# Autodesk Inventor assembly: EngineComplete
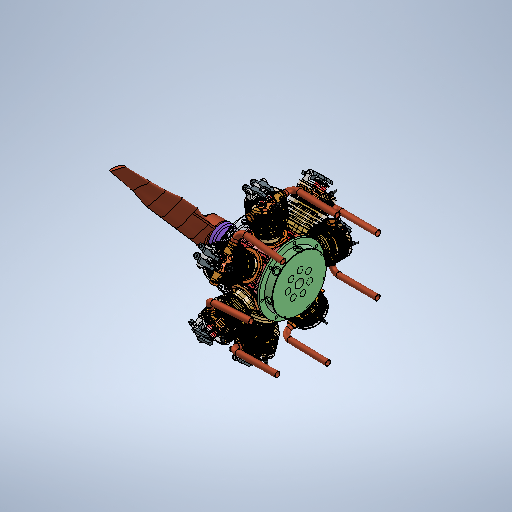
[picture p0: Inventor's stored thumbnail of the model, 512x512]
Saved by Autodesk Inventor 2025 (Build 290162010, 162A)
## iProperties
Created: 2024-07-16
Part Number: EngineComplete
Document SubType Name: Assembly
Designer: ffogue
Author: ffogue
## Documents named in this file (15)
- C:\Users\Fabri\Documents\Inventor\Stermotor\EngineComplete.iam
- C:\Users\Fabri\Documents\Inventor\Stermotor\Zylinder.ipt
- C:\Users\Fabri\Documents\Inventor\Stermotor\MotorBlock_First.iam
- C:\Users\Fabri\Documents\Inventor\Stermotor\pleuel.ipt
- C:\Users\Fabri\Documents\Inventor\Stermotor\Kolben.iam
- C:\Users\Fabri\Documents\Inventor\Stermotor\MotorBlock.iam
- C:\Users\Fabri\Documents\Inventor\Stermotor\sonnenrad.ipt
- C:\Users\Fabri\Documents\Inventor\Stermotor\Decke_grün.ipt
- C:\Users\Fabri\Documents\Inventor\Stermotor\Cylinder.iam
- C:\Users\Fabri\Documents\Inventor\Stermotor\VenturiEinsatz.ipt
- C:\Users\Fabri\Documents\Inventor\Stermotor\zylinderfussdichtung.ipt
- C:\Users\Fabri\Documents\Inventor\Stermotor\Aschse.iam
- C:\Users\Fabri\Documents\Inventor\Stermotor\PlanetenRad.ipt
- C:\Users\Fabri\Documents\Inventor\Stermotor\Stirnzahnrad12.ipt
- C:\Users\Fabri\Documents\Inventor\Stermotor\Rad16_5.ipt
## Components (47 placed, 13 different names)
1. Zylinder:1 — Mate:1, Mate:2, Insert:1, Mate:4, Mate:8, Mate:10, Mate:11, Mate:12, Mate:13, Insert:10, Mate:30, Insert:14, Mate:39, Insert:18, Insert:19, Insert:20, Insert:21, Insert:22, Insert:23, Mate:50, Insert:28
2. MotorBlock_First:1 [sub-assembly] — Mate:2, Insert:1, Mate:5, Insert:2, Mate:7, Insert:3, Mate:14, Insert:4, Mate:16, Insert:5, Mate:18, Insert:6, Mate:20, Insert:7, Mate:28, Insert:12, Insert:29
3. Kolben:1 [sub-assembly] — Mate:4, Mate:6, Mate:26
4. pleuel:1 — Mate:5, Insert:2, Mate:6
5. pleuel:3 — Mate:7, Insert:3, Mate:9
6. Kolben:3 [sub-assembly] — Mate:8, Mate:9, Mate:44
7. Kolben:4 [sub-assembly] — Mate:10, Mate:15, Mate:43
8. Kolben:5 [sub-assembly] — Mate:11, Mate:17, Mate:42
9. Kolben:6 [sub-assembly] — Mate:12, Mate:19, Mate:41
10. Kolben:7 [sub-assembly] — Mate:13, Mate:21, Mate:40
11. pleuel:4 — Mate:14, Mate:15, Insert:4
12. pleuel:5 — Mate:16, Mate:17, Insert:5
13. pleuel:6 — Mate:18, Insert:6, Mate:19
14. pleuel:7 — Mate:20, Insert:7, Mate:21
15. sonnenrad:1 — Mate:30, Insert:14, Mate:38
16. Decke_grün:1 — Mate:34, Mate:38, Mate:39, Insert:17, Insert:18, Mate:53
17. MotorBlock:2 [sub-assembly] — Mate:28, Insert:12
18. MotorBlock:1 [sub-assembly] — Mate:27, Insert:11
19. Cylinder:1 [sub-assembly] — Mate:26, Mate:27, Insert:10, Insert:11
20. Cylinder:2 [sub-assembly] — Mate:40, Insert:19, Mate:45, Insert:24
21. Cylinder:3 [sub-assembly] — Mate:41, Insert:20, Mate:46, Insert:25
22. Cylinder:4 [sub-assembly] — Mate:42, Insert:21, Mate:47, Insert:26
23. Cylinder:5 [sub-assembly] — Mate:43, Insert:22, Mate:48, Insert:27
24. Cylinder:6 [sub-assembly] — Mate:44, Insert:23, Mate:49
25. MotorBlock:3 [sub-assembly] — Mate:49
26. MotorBlock:4 [sub-assembly] — Mate:48, Insert:27
27. MotorBlock:5 [sub-assembly] — Mate:47, Insert:26
28. MotorBlock:6 [sub-assembly] — Mate:46, Insert:25
29. MotorBlock:7 [sub-assembly] — Mate:45, Insert:24
30. Aschse:1 [sub-assembly] — Rotation:2, Mate:53, Insert:29, Mate:54, Insert:30
31. Stirnzahnrad1:1 — Mate:52, Flush:1, Rotation:1, Flush:2, Rotation:4
32. Stirnzahnrad1:2 — Mate:52, Flush:1, Rotation:1, Rotation:2, Main Motion, Rotation:3, Tangent:2, Mate:54, Insert:30
33. Stirnzahnrad2:1 — Flush:2, Rotation:3, Tangent:2, Rotation:4
34. VenturiEinsatz:2 — Mate:34, Insert:17
35. VenturiEinsatz:3
36. VenturiEinsatz:4
37. VenturiEinsatz:5
38. VenturiEinsatz:6
39. VenturiEinsatz:7
40. VenturiEinsatz:8
41. zylinderfussdichtung:1 — Mate:50, Insert:28
42. zylinderfussdichtung:2
43. zylinderfussdichtung:3
44. zylinderfussdichtung:4
45. zylinderfussdichtung:5
46. zylinderfussdichtung:6
47. zylinderfussdichtung:7
## Component patterns: (7 elements, first: VenturiEinsatz:2), (7 elements, first: zylinderfussdichtung:1)
## Relationships (74: Mate 41, Insert 25, RelateRotation 4, Flush 2, Angle 1, Tangent 1)
- Mate:1: Zylinder:1
- Mate:2: Zylinder:1 ↔ MotorBlock_First:1
- Insert:1: Zylinder:1 ↔ MotorBlock_First:1
- Mate:4: Zylinder:1 ↔ Kolben:1
- Mate:5: MotorBlock_First:1 ↔ pleuel:1
- Insert:2: MotorBlock_First:1 ↔ pleuel:1
- Mate:6: Kolben:1 ↔ pleuel:1
- Mate:7: MotorBlock_First:1 ↔ pleuel:3
- Insert:3: MotorBlock_First:1 ↔ pleuel:3
- Mate:8: Zylinder:1 ↔ Kolben:3
- Mate:9: pleuel:3 ↔ Kolben:3
- Mate:10: Zylinder:1 ↔ Kolben:4
- Mate:11: Zylinder:1 ↔ Kolben:5
- Mate:12: Zylinder:1 ↔ Kolben:6
- Mate:13: Zylinder:1 ↔ Kolben:7
- Mate:14: MotorBlock_First:1 ↔ pleuel:4
- Mate:15: Kolben:4 ↔ pleuel:4
- Insert:4: MotorBlock_First:1 ↔ pleuel:4
- Mate:16: MotorBlock_First:1 ↔ pleuel:5
- Mate:17: Kolben:5 ↔ pleuel:5
- Insert:5: MotorBlock_First:1 ↔ pleuel:5
- Mate:18: MotorBlock_First:1 ↔ pleuel:6
- Insert:6: MotorBlock_First:1 ↔ pleuel:6
- Mate:19: Kolben:6 ↔ pleuel:6
- Mate:20: MotorBlock_First:1 ↔ pleuel:7
- Insert:7: MotorBlock_First:1 ↔ pleuel:7
- Mate:21: Kolben:7 ↔ pleuel:7
- Mate:26: Kolben:1 ↔ Cylinder:1
- Mate:27: MotorBlock:1 ↔ Cylinder:1
- Insert:10 (-5.5 mm): Zylinder:1 ↔ Cylinder:1
- Insert:11: MotorBlock:1 ↔ Cylinder:1
- Mate:28: MotorBlock_First:1 ↔ MotorBlock:2
- Insert:12: MotorBlock_First:1 ↔ MotorBlock:2
- Mate:30: Zylinder:1 ↔ sonnenrad:1
- Insert:14: Zylinder:1 ↔ sonnenrad:1
- Mate:34: Decke_grün:1 ↔ VenturiEinsatz:2
- Mate:38: sonnenrad:1 ↔ Decke_grün:1
- Mate:39: Zylinder:1 ↔ Decke_grün:1
- Insert:17: Decke_grün:1 ↔ VenturiEinsatz:2
- Insert:18: Zylinder:1 ↔ Decke_grün:1
- Mate:40: Kolben:7 ↔ Cylinder:2
- Insert:19 (-5.5 mm): Zylinder:1 ↔ Cylinder:2
- Mate:41: Kolben:6 ↔ Cylinder:3
- Insert:20 (-5.5 mm): Zylinder:1 ↔ Cylinder:3
- Mate:42: Kolben:5 ↔ Cylinder:4
- Insert:21 (-5.5 mm): Zylinder:1 ↔ Cylinder:4
- Mate:43: Kolben:4 ↔ Cylinder:5
- Insert:22 (-5.5 mm): Zylinder:1 ↔ Cylinder:5
- Mate:44: Kolben:3 ↔ Cylinder:6
- Insert:23 (-5.5 mm): Zylinder:1 ↔ Cylinder:6
- Mate:45: Cylinder:2 ↔ MotorBlock:7
- Insert:24: Cylinder:2 ↔ MotorBlock:7
- Mate:46: Cylinder:3 ↔ MotorBlock:6
- Insert:25: Cylinder:3 ↔ MotorBlock:6
- Mate:47: Cylinder:4 ↔ MotorBlock:5
- Insert:26: Cylinder:4 ↔ MotorBlock:5
- Mate:48: Cylinder:5 ↔ MotorBlock:4
- Insert:27: Cylinder:5 ↔ MotorBlock:4
- Mate:49: Cylinder:6 ↔ MotorBlock:3
- Mate:50: Zylinder:1 ↔ zylinderfussdichtung:1
- Insert:28: Zylinder:1 ↔ zylinderfussdichtung:1
- Mate:52: Stirnzahnrad1:1 ↔ Stirnzahnrad1:2
- Flush:1: Stirnzahnrad1:1 ↔ Stirnzahnrad1:2
- Rotation:1 [RelateRotation] (0.4783 ul): Stirnzahnrad1:1 ↔ Stirnzahnrad1:2
- Rotation:2 [RelateRotation] (1 ul): Aschse:1 ↔ Stirnzahnrad1:2
- Main Motion [Angle] (0 deg): Stirnzahnrad1:2
- Flush:2: Stirnzahnrad1:1 ↔ Stirnzahnrad2:1
- Rotation:3 [RelateRotation] (0.5 ul): Stirnzahnrad1:2 ↔ Stirnzahnrad2:1
- Tangent:2: Stirnzahnrad1:2 ↔ Stirnzahnrad2:1
- Rotation:4 [RelateRotation] (0.2391 ul): Stirnzahnrad1:1 ↔ Stirnzahnrad2:1
- Mate:53: Decke_grün:1 ↔ Aschse:1
- Insert:29: MotorBlock_First:1 ↔ Aschse:1
- Mate:54: Aschse:1 ↔ Stirnzahnrad1:2
- Insert:30: Aschse:1 ↔ Stirnzahnrad1:2
